# Autodesk Inventor assembly: Pool House
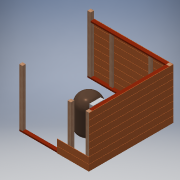
[picture p0: Inventor's stored thumbnail of the model, 180x180]
Saved by Autodesk Inventor 2016 (Build 200138000, 138)
## iProperties
Created: 2015-05-30
Part Number: Pool House
Document SubType Name: Assembly
Designer: steele
Author: steele
## Documents named in this file (17)
- C:\FRC\FMHS-CAD\Steele House Project\Pool House.iam
- C:\FRC\FMHS-CAD\Steele House Project\Base for Pool House.ipt
- C:\FRC\FMHS-CAD\Steele House Project\Front Post North Side.ipt
- C:\FRC\FMHS-CAD\Steele House Project\Front Post South Side.ipt
- C:\FRC\FMHS-CAD\Steele House Project\Rear Post North Side.ipt
- C:\FRC\FMHS-CAD\Steele House Project\Rear Post South Side.ipt
- C:\FRC\FMHS-CAD\Steele House Project\Pool Controller.ipt
- C:\FRC\FMHS-CAD\Steele House Project\Home Depot Composite Slat 69 in.ipt
- C:\FRC\FMHS-CAD\Steele House Project\Home Depot Composite Slat 19_75 in.ipt
- C:\FRC\FMHS-CAD\Steele House Project\Lumber 2x4x82.ipt
- C:\FRC\FMHS-CAD\Steele House Project\Home Depot Composite Slat 22_75 in.ipt
- C:\FRC\FMHS-CAD\Steele House Project\Home Depot Composite Slat 64 7_16 in.ipt
- C:\FRC\FMHS-CAD\Steele House Project\Lumbwer 2x4x50_75.ipt
- C:\FRC\FMHS-CAD\Steele House Project\Lumber 2x4x80.ipt
- C:\FRC\FMHS-CAD\Steele House Project\Pool Filter.ipt
- C:\FRC\FMHS-CAD\Steele House Project\Home Depot Composite Slat 34 in.ipt
- C:\FRC\FMHS-CAD\Steele House Project\Molding 4 ft.ipt
## Components (49 placed, 16 different names)
1. Base for Pool House:1 — Mate:1, Flush:1, Flush:2, Mate:2, Flush:3, Flush:4, Mate:3, Flush:5, Flush:6, Mate:4, Flush:7, Flush:8, Mate:8, Flush:11, Mate:9, Mate:10, Flush:21, Flush:22, Mate:77, Mate:79, Mate:82, Flush:32, Mate:84, Flush:33, Flush:34, Tangent:1, Tangent:2, Mate:86, Flush:35, Flush:36, Flush:37
2. Front Post North Side:1 — Mate:1, Flush:1, Flush:2, Mate:5, Flush:9, Flush:10, Mate:11, Mate:12, Mate:13, Mate:20, Mate:24, Mate:28, Mate:32, Mate:38, Mate:40, Mate:78
3. Front Post South Side:1 — Mate:2, Flush:3, Flush:4, Mate:7, Mate:15, Mate:22, Mate:27, Mate:30, Mate:34, Mate:36, Mate:42, Mate:80, Mate:81, Flush:30, Flush:31, Mate:85
4. Rear Post North Side:1 — Mate:3, Flush:5, Flush:6, Mate:87
5. Rear Post South Side:1 — Mate:4, Flush:7, Flush:8, Mate:45, Mate:47, Mate:53, Mate:55, Mate:61, Mate:69, Mate:71, Mate:75, Mate:83
6. Pool Controller:1 — Mate:5, Flush:9, Flush:10
7. Home Depot Composite Slat 69 in:1 — Mate:7, Mate:8, Flush:11, Mate:16, Flush:14, Mate:46
8. Home Depot Composite Slat 19_75 in:1 — Mate:9, Mate:10, Mate:14, Flush:14, Mate:88
9. Lumber 2x4x82:1 — Mate:11, Mate:12
10. Home Depot Composite Slat 69 in:2 — Mate:13, Mate:14, Mate:21, Mate:23, Flush:13, Mate:89
11. Home Depot Composite Slat 19_75 in:2 — Mate:15, Mate:16, Flush:13, Mate:49
12. Home Depot Composite Slat 69 in:3 — Mate:22, Mate:23, Flush:12, Mate:26, Mate:51
13. Home Depot Composite Slat 19_75 in:3 — Mate:20, Mate:21, Flush:12, Mate:25
14. Home Depot Composite Slat 69 in:4 — Mate:24, Mate:25, Flush:15, Mate:29
15. Home Depot Composite Slat 19_75 in:4 — Mate:26, Mate:27, Flush:15, Mate:31, Mate:57
16. Home Depot Composite Slat 19_75 in:5 — Mate:28, Mate:29, Flush:16
17. Home Depot Composite Slat 69 in:5 — Mate:30, Mate:31, Flush:16, Mate:33, Mate:35, Mate:59
18. Home Depot Composite Slat 69 in:6 — Mate:32, Mate:33, Flush:17, Mate:39
19. Home Depot Composite Slat 19_75 in:6 — Mate:34, Mate:35, Flush:17, Mate:37, Flush:29
20. Home Depot Composite Slat 69 in:7 — Mate:36, Mate:37, Flush:18, Mate:41, Mate:43, Mate:65, Flush:29
21. Home Depot Composite Slat 19_75 in:7 — Mate:38, Mate:39, Flush:18
22. Home Depot Composite Slat 69 in:8 — Mate:40, Mate:41, Flush:19
23. Home Depot Composite Slat 19_75 in:8 — Mate:42, Mate:43, Flush:19, Mate:67, Mate:73
24. Home Depot Composite Slat 22_75 in:1 — Mate:45, Flush:21, Mate:48, Flush:23
25. Home Depot Composite Slat 64 7_16 in:1 — Mate:46, Flush:22, Flush:23, Mate:50
26. Home Depot Composite Slat 64 7_16 in:2 — Mate:47, Mate:48, Flush:24, Mate:54
27. Home Depot Composite Slat 22_75 in:2 — Mate:49, Mate:50, Flush:24, Mate:52
28. Home Depot Composite Slat 64 7_16 in:3 — Mate:51, Mate:52, Flush:25, Mate:58
29. Home Depot Composite Slat 22_75 in:3 — Mate:53, Mate:54, Flush:25, Mate:56
30. Home Depot Composite Slat 64 7_16 in:4 — Mate:55, Mate:56, Flush:26, Mate:62
31. Home Depot Composite Slat 22_75 in:4 — Mate:57, Mate:58, Flush:26, Mate:60
32. Home Depot Composite Slat 64 7_16 in:5 — Mate:59, Mate:60, Flush:27, Mate:64, Mate:70
33. Home Depot Composite Slat 64 7_16 in:6 — Mate:64, Mate:69, Flush:28, Mate:72
34. Home Depot Composite Slat 64 7_16 in:7 — Mate:67, Mate:68, Mate:74, Mate:76
35. Home Depot Composite Slat 22_75 in:5 — Mate:61, Mate:62, Flush:27
36. Home Depot Composite Slat 22_75 in:6 — Mate:65, Mate:68, Mate:70, Flush:28
37. Home Depot Composite Slat 22_75 in:7 — Mate:71, Mate:72
38. Home Depot Composite Slat 22_75 in:8 — Mate:73, Mate:74, Mate:91
39. Home Depot Composite Slat 64 7_16 in:8 — Mate:75, Mate:76
40. Lumbwer 2x4x50_75:1 — Mate:77, Mate:78
41. Lumbwer 2x4x50_75:2 — Mate:79, Mate:80
42. Lumber 2x4x80:1 — Mate:81, Flush:30, Flush:31
43. Lumbwer 2x4x50_75:3 — Mate:82, Mate:83, Flush:32
44. Lumbwer 2x4x50_75:4 — Mate:84, Mate:85, Flush:33
45. Pool Filter:1 — Flush:34, Tangent:1, Tangent:2
46. Front Post North Side:2 — Mate:86, Flush:35, Mate:87
47. Home Depot Composite Slat 34 in:1 — Mate:88, Flush:36, Mate:90
48. Home Depot Composite Slat 34 in:2 — Mate:89, Mate:90
49. Molding 4 ft:1 — Mate:91, Flush:37
## Relationships (122: Mate 84, Flush 36, Tangent 2)
- Mate:1: Base for Pool House:1 ↔ Front Post North Side:1
- Flush:1: Base for Pool House:1 ↔ Front Post North Side:1
- Flush:2: Base for Pool House:1 ↔ Front Post North Side:1
- Mate:2: Base for Pool House:1 ↔ Front Post South Side:1
- Flush:3: Base for Pool House:1 ↔ Front Post South Side:1
- Flush:4: Base for Pool House:1 ↔ Front Post South Side:1
- Mate:3: Base for Pool House:1 ↔ Rear Post North Side:1
- Flush:5: Base for Pool House:1 ↔ Rear Post North Side:1
- Flush:6: Base for Pool House:1 ↔ Rear Post North Side:1
- Mate:4: Base for Pool House:1 ↔ Rear Post South Side:1
- Flush:7: Base for Pool House:1 ↔ Rear Post South Side:1
- Flush:8: Base for Pool House:1 ↔ Rear Post South Side:1
- Mate:5 (127 mm): Front Post North Side:1 ↔ Pool Controller:1
- Flush:9: Front Post North Side:1 ↔ Pool Controller:1
- Flush:10 (101.6 mm): Front Post North Side:1 ↔ Pool Controller:1
- Mate:7: Front Post South Side:1 ↔ Home Depot Composite Slat 69 in:1
- Mate:8: Base for Pool House:1 ↔ Home Depot Composite Slat 69 in:1
- Flush:11: Base for Pool House:1 ↔ Home Depot Composite Slat 69 in:1
- Mate:9: Base for Pool House:1 ↔ Home Depot Composite Slat 19_75 in:1
- Mate:10: Base for Pool House:1 ↔ Home Depot Composite Slat 19_75 in:1
- Mate:11: Front Post North Side:1 ↔ Lumber 2x4x82:1
- Mate:12: Front Post North Side:1 ↔ Lumber 2x4x82:1
- Mate:13: Front Post North Side:1 ↔ Home Depot Composite Slat 69 in:2
- Mate:14 (6.35 mm): Home Depot Composite Slat 19_75 in:1 ↔ Home Depot Composite Slat 69 in:2
- Mate:15: Front Post South Side:1 ↔ Home Depot Composite Slat 19_75 in:2
- Mate:16 (6.35 mm): Home Depot Composite Slat 69 in:1 ↔ Home Depot Composite Slat 19_75 in:2
- Mate:20: Front Post North Side:1 ↔ Home Depot Composite Slat 19_75 in:3
- Mate:21 (6.35 mm): Home Depot Composite Slat 69 in:2 ↔ Home Depot Composite Slat 19_75 in:3
- Mate:22: Front Post South Side:1 ↔ Home Depot Composite Slat 69 in:3
- Mate:23 (6.35 mm): Home Depot Composite Slat 69 in:2 ↔ Home Depot Composite Slat 69 in:3
- Flush:12: Home Depot Composite Slat 69 in:3 ↔ Home Depot Composite Slat 19_75 in:3
- Flush:13: Home Depot Composite Slat 69 in:2 ↔ Home Depot Composite Slat 19_75 in:2
- Flush:14: Home Depot Composite Slat 69 in:1 ↔ Home Depot Composite Slat 19_75 in:1
- Mate:24: Front Post North Side:1 ↔ Home Depot Composite Slat 69 in:4
- Mate:25 (6.35 mm): Home Depot Composite Slat 19_75 in:3 ↔ Home Depot Composite Slat 69 in:4
- Mate:26 (6.35 mm): Home Depot Composite Slat 69 in:3 ↔ Home Depot Composite Slat 19_75 in:4
- Mate:27: Front Post South Side:1 ↔ Home Depot Composite Slat 19_75 in:4
- Flush:15: Home Depot Composite Slat 69 in:4 ↔ Home Depot Composite Slat 19_75 in:4
- Mate:28: Front Post North Side:1 ↔ Home Depot Composite Slat 19_75 in:5
- Mate:29 (6.35 mm): Home Depot Composite Slat 69 in:4 ↔ Home Depot Composite Slat 19_75 in:5
- Mate:30: Front Post South Side:1 ↔ Home Depot Composite Slat 69 in:5
- Mate:31 (6.35 mm): Home Depot Composite Slat 19_75 in:4 ↔ Home Depot Composite Slat 69 in:5
- Flush:16: Home Depot Composite Slat 19_75 in:5 ↔ Home Depot Composite Slat 69 in:5
- Mate:32: Front Post North Side:1 ↔ Home Depot Composite Slat 69 in:6
- Mate:33 (6.35 mm): Home Depot Composite Slat 69 in:5 ↔ Home Depot Composite Slat 69 in:6
- Mate:34: Front Post South Side:1 ↔ Home Depot Composite Slat 19_75 in:6
- Mate:35 (6.35 mm): Home Depot Composite Slat 69 in:5 ↔ Home Depot Composite Slat 19_75 in:6
- Flush:17: Home Depot Composite Slat 69 in:6 ↔ Home Depot Composite Slat 19_75 in:6
- Mate:36: Front Post South Side:1 ↔ Home Depot Composite Slat 69 in:7
- Mate:37 (6.35 mm): Home Depot Composite Slat 19_75 in:6 ↔ Home Depot Composite Slat 69 in:7
- Mate:38: Front Post North Side:1 ↔ Home Depot Composite Slat 19_75 in:7
- Mate:39 (6.35 mm): Home Depot Composite Slat 69 in:6 ↔ Home Depot Composite Slat 19_75 in:7
- Flush:18: Home Depot Composite Slat 69 in:7 ↔ Home Depot Composite Slat 19_75 in:7
- Mate:40: Front Post North Side:1 ↔ Home Depot Composite Slat 69 in:8
- Mate:41 (6.35 mm): Home Depot Composite Slat 69 in:7 ↔ Home Depot Composite Slat 69 in:8
- Mate:42: Front Post South Side:1 ↔ Home Depot Composite Slat 19_75 in:8
- Mate:43 (6.35 mm): Home Depot Composite Slat 69 in:7 ↔ Home Depot Composite Slat 19_75 in:8
- Flush:19: Home Depot Composite Slat 69 in:8 ↔ Home Depot Composite Slat 19_75 in:8
- Mate:45: Rear Post South Side:1 ↔ Home Depot Composite Slat 22_75 in:1
- Flush:21: Base for Pool House:1 ↔ Home Depot Composite Slat 22_75 in:1
- Mate:46: Home Depot Composite Slat 69 in:1 ↔ Home Depot Composite Slat 64 7_16 in:1
- Flush:22: Base for Pool House:1 ↔ Home Depot Composite Slat 64 7_16 in:1
- Mate:47: Rear Post South Side:1 ↔ Home Depot Composite Slat 64 7_16 in:2
- Mate:48 (6.35 mm): Home Depot Composite Slat 22_75 in:1 ↔ Home Depot Composite Slat 64 7_16 in:2
- Flush:23: Home Depot Composite Slat 22_75 in:1 ↔ Home Depot Composite Slat 64 7_16 in:1
- Mate:49: Home Depot Composite Slat 19_75 in:2 ↔ Home Depot Composite Slat 22_75 in:2
- Mate:50 (6.35 mm): Home Depot Composite Slat 64 7_16 in:1 ↔ Home Depot Composite Slat 22_75 in:2
- Flush:24: Home Depot Composite Slat 64 7_16 in:2 ↔ Home Depot Composite Slat 22_75 in:2
- Mate:51: Home Depot Composite Slat 69 in:3 ↔ Home Depot Composite Slat 64 7_16 in:3
- Mate:52 (6.35 mm): Home Depot Composite Slat 22_75 in:2 ↔ Home Depot Composite Slat 64 7_16 in:3
- Mate:53: Rear Post South Side:1 ↔ Home Depot Composite Slat 22_75 in:3
- Mate:54 (6.35 mm): Home Depot Composite Slat 64 7_16 in:2 ↔ Home Depot Composite Slat 22_75 in:3
- Flush:25: Home Depot Composite Slat 64 7_16 in:3 ↔ Home Depot Composite Slat 22_75 in:3
- Mate:55: Rear Post South Side:1 ↔ Home Depot Composite Slat 64 7_16 in:4
- Mate:56 (6.35 mm): Home Depot Composite Slat 22_75 in:3 ↔ Home Depot Composite Slat 64 7_16 in:4
- Mate:57: Home Depot Composite Slat 19_75 in:4 ↔ Home Depot Composite Slat 22_75 in:4
- Mate:58 (6.35 mm): Home Depot Composite Slat 64 7_16 in:3 ↔ Home Depot Composite Slat 22_75 in:4
- Flush:26: Home Depot Composite Slat 64 7_16 in:4 ↔ Home Depot Composite Slat 22_75 in:4
- Mate:59: Home Depot Composite Slat 69 in:5 ↔ Home Depot Composite Slat 64 7_16 in:5
- Mate:60 (6.35 mm): Home Depot Composite Slat 22_75 in:4 ↔ Home Depot Composite Slat 64 7_16 in:5
- Mate:61: Rear Post South Side:1 ↔ Home Depot Composite Slat 22_75 in:5
- Mate:62 (6.35 mm): Home Depot Composite Slat 64 7_16 in:4 ↔ Home Depot Composite Slat 22_75 in:5
- Flush:27: Home Depot Composite Slat 64 7_16 in:5 ↔ Home Depot Composite Slat 22_75 in:5
- Mate:64 (6.35 mm): Home Depot Composite Slat 64 7_16 in:5 ↔ Home Depot Composite Slat 64 7_16 in:6
- Mate:65: Home Depot Composite Slat 69 in:7 ↔ Home Depot Composite Slat 22_75 in:6
- Mate:67: Home Depot Composite Slat 19_75 in:8 ↔ Home Depot Composite Slat 64 7_16 in:7
- Mate:68 (6.35 mm): Home Depot Composite Slat 64 7_16 in:7 ↔ Home Depot Composite Slat 22_75 in:6
- Mate:69: Rear Post South Side:1 ↔ Home Depot Composite Slat 64 7_16 in:6
- Mate:70 (6.35 mm): Home Depot Composite Slat 64 7_16 in:5 ↔ Home Depot Composite Slat 22_75 in:6
- Flush:28: Home Depot Composite Slat 64 7_16 in:6 ↔ Home Depot Composite Slat 22_75 in:6
- Flush:29: Home Depot Composite Slat 19_75 in:6 ↔ Home Depot Composite Slat 69 in:7
- Mate:71: Rear Post South Side:1 ↔ Home Depot Composite Slat 22_75 in:7
- Mate:72 (6.35 mm): Home Depot Composite Slat 64 7_16 in:6 ↔ Home Depot Composite Slat 22_75 in:7
- Mate:73: Home Depot Composite Slat 19_75 in:8 ↔ Home Depot Composite Slat 22_75 in:8
- Mate:74 (6.35 mm): Home Depot Composite Slat 64 7_16 in:7 ↔ Home Depot Composite Slat 22_75 in:8
- Mate:75: Rear Post South Side:1 ↔ Home Depot Composite Slat 64 7_16 in:8
- Mate:76 (6.35 mm): Home Depot Composite Slat 64 7_16 in:7 ↔ Home Depot Composite Slat 64 7_16 in:8
- Mate:77: Base for Pool House:1 ↔ Lumbwer 2x4x50_75:1
- Mate:78 (371.475 mm): Front Post North Side:1 ↔ Lumbwer 2x4x50_75:1
- Mate:79: Base for Pool House:1 ↔ Lumbwer 2x4x50_75:2
- Mate:80 (371.475 mm): Front Post South Side:1 ↔ Lumbwer 2x4x50_75:2
- Mate:81: Front Post South Side:1 ↔ Lumber 2x4x80:1
- Flush:30: Front Post South Side:1 ↔ Lumber 2x4x80:1
- Flush:31: Front Post South Side:1 ↔ Lumber 2x4x80:1
- Mate:82: Base for Pool House:1 ↔ Lumbwer 2x4x50_75:3
- Mate:83 (447.5607 mm): Rear Post South Side:1 ↔ Lumbwer 2x4x50_75:3
- Flush:32: Base for Pool House:1 ↔ Lumbwer 2x4x50_75:3
- Mate:84: Base for Pool House:1 ↔ Lumbwer 2x4x50_75:4
- Mate:85 (436.5625 mm): Front Post South Side:1 ↔ Lumbwer 2x4x50_75:4
- Flush:33: Base for Pool House:1 ↔ Lumbwer 2x4x50_75:4
- Flush:34: Base for Pool House:1 ↔ Pool Filter:1
- Tangent:1 (609.6 mm): Base for Pool House:1 ↔ Pool Filter:1
- Tangent:2 (609.6 mm): Base for Pool House:1 ↔ Pool Filter:1
- Mate:86: Base for Pool House:1 ↔ Front Post North Side:2
- Flush:35: Base for Pool House:1 ↔ Front Post North Side:2
- Mate:87 (1219.2 mm): Rear Post North Side:1 ↔ Front Post North Side:2
- Mate:88: Home Depot Composite Slat 19_75 in:1 ↔ Home Depot Composite Slat 34 in:1
- Flush:36: Base for Pool House:1 ↔ Home Depot Composite Slat 34 in:1
- Mate:89: Home Depot Composite Slat 69 in:2 ↔ Home Depot Composite Slat 34 in:2
- Mate:90 (6.35 mm): Home Depot Composite Slat 34 in:1 ↔ Home Depot Composite Slat 34 in:2
- Mate:91: Home Depot Composite Slat 22_75 in:8 ↔ Molding 4 ft:1
- Flush:37: Base for Pool House:1 ↔ Molding 4 ft:1
